# Autodesk Inventor assembly: Ensamblaje_soportme molde_barras
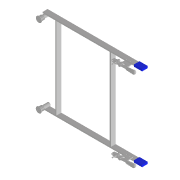
[picture p0: Inventor's stored thumbnail of the model, 180x180]
Saved by Autodesk Inventor 2021 (Build 250183000, 183)
## iProperties
Created: 2021-04-17
Part Number: Ensamblaje_soportme molde_barras
Document SubType Name: Assembly
Designer: Admin
Author: Admin
## Documents named in this file (7)
- C:\Users\carlo\Desktop\Pai\Proyecto_PAI_2021\01 CAD\Ensamblaje_soportme molde_barras.iam
- C:\Users\carlo\Desktop\Pai\Proyecto_PAI_2021\01 CAD\Soporte_molde.ipt
- C:\Users\carlo\Desktop\Pai\Proyecto_PAI_2021\01 CAD\Mangas_soporte_molde.ipt
- C:\Users\carlo\Desktop\Pai\Proyecto_PAI_2021\01 CAD\Toggle_clamp.iam
- C:\Users\carlo\Desktop\Pai\Proyecto_PAI_2021\01 CAD\Barra_circular_soporte.ipt
- C:\Users\carlo\Desktop\Pai\Proyecto_PAI_2021\01 CAD\Pasador_soporte.ipt
- C:\Users\carlo\Desktop\Pai\Proyecto_PAI_2021\01 CAD\Resorte_soporte_ material.ipt
## Components (11 placed, 6 different names)
1. Soporte_molde:1 — Coincidencia:1, Coincidencia:2, Coincidencia:3, Coincidencia:4, Coincidencia:5, Coincidencia:6, Coincidencia:7, Coincidencia:8, De rotación:1, De rotación:2
2. Mangas_soporte_molde:1 — Coincidencia:1, Coincidencia:2, Coincidencia:3
3. Mangas_soporte_molde:2 — Coincidencia:4, Coincidencia:5, Coincidencia:6
4. Toggle_clamp:1 [sub-assembly] — Coincidencia:7
5. Toggle_clamp:2 [sub-assembly] — Coincidencia:8
6. Barra_circular_soporte:1 — De rotación:1, Coincidencia:9, Nivelación:1, Coincidencia:11
7. Barra_circular_soporte:2 — De rotación:2, Coincidencia:10, Nivelación:2, Coincidencia:12
8. Pasador_soporte:1 — Coincidencia:9, Nivelación:1, Tangente:1
9. Pasador_soporte:2 — Coincidencia:10, Nivelación:2, Tangente:2
10. Resorte_soporte_ material:1 — Coincidencia:12, Tangente:2
11. Resorte_soporte_ material:2 — Coincidencia:11, Tangente:1
## Relationships (18: Mate 12, RevoluteJoint 2, Flush 2, Tangent 2)
- Coincidencia:1 [Mate]: Soporte_molde:1 ↔ Mangas_soporte_molde:1
- Coincidencia:2 [Mate]: Soporte_molde:1 ↔ Mangas_soporte_molde:1
- Coincidencia:3 [Mate]: Soporte_molde:1 ↔ Mangas_soporte_molde:1
- Coincidencia:4 [Mate]: Soporte_molde:1 ↔ Mangas_soporte_molde:2
- Coincidencia:5 [Mate]: Soporte_molde:1 ↔ Mangas_soporte_molde:2
- Coincidencia:6 [Mate]: Soporte_molde:1 ↔ Mangas_soporte_molde:2
- Coincidencia:7 [Mate]: Soporte_molde:1 ↔ Toggle_clamp:1
- Coincidencia:8 [Mate]: Soporte_molde:1 ↔ Toggle_clamp:2
- De rotación:1 [RevoluteJoint]: Soporte_molde:1 ↔ Barra_circular_soporte:1
- De rotación:2 [RevoluteJoint]: Soporte_molde:1 ↔ Barra_circular_soporte:2
- Coincidencia:9 [Mate]: Barra_circular_soporte:1 ↔ Pasador_soporte:1
- Nivelación:1 [Flush]: Barra_circular_soporte:1 ↔ Pasador_soporte:1
- Coincidencia:10 [Mate]: Barra_circular_soporte:2 ↔ Pasador_soporte:2
- Nivelación:2 [Flush]: Barra_circular_soporte:2 ↔ Pasador_soporte:2
- Coincidencia:11 [Mate]: Barra_circular_soporte:1 ↔ Resorte_soporte_ material:2
- Tangente:1: Pasador_soporte:1 ↔ Resorte_soporte_ material:2
- Coincidencia:12 [Mate]: Barra_circular_soporte:2 ↔ Resorte_soporte_ material:1
- Tangente:2: Pasador_soporte:2 ↔ Resorte_soporte_ material:1
